# Autodesk Inventor assembly: Montagem1
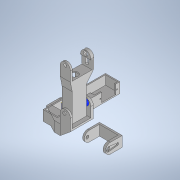
[picture p0: Inventor's stored thumbnail of the model, 180x180]
Saved by Autodesk Inventor 2022.2 (Build 262287010, 287A)
## iProperties
Created: 2022-04-04
Part Number: Montagem1
Document SubType Name: Assembly
Designer: nakai
Author: nakai
## Documents named in this file (7)
- C:\Users\nakai\Dropbox\reprap\Robo dog mini\Montagem1.iam
- C:\Users\nakai\Dropbox\reprap\Robo dog mini\ombro_base.ipt
- C:\Users\nakai\Dropbox\reprap\Robo dog mini\ombro_dir.ipt
- C:\Users\nakai\Dropbox\reprap\Robo dog mini\ombro_esq.ipt
- C:\Users\nakai\Dropbox\reprap\Robo dog mini\corpo.ipt
- C:\Users\nakai\Dropbox\reprap\Robo dog mini\servo_motor.ipt
- C:\Users\nakai\Dropbox\reprap\Robo dog mini\perna_esq.ipt
## Components (7 placed, 6 different names)
1. ombro_base:1 — Inserir:3, Inserir:4, Inserir:5
2. ombro_dir:1
3. ombro_esq:1 — Inserir:4, Inserir:5, Rotativa:1
4. corpo:1 — Inserir:1, Inserir:2, Inserir:3
5. servo_motor:1 — Inserir:1, Inserir:2
6. perna_esq:1 — Inserir:6, Inserir:7, Rotativa:1
7. servo_motor:2 — Inserir:6, Inserir:7
## Relationships (8: Insert 7, RevoluteJoint 1)
- Inserir:1: corpo:1 ↔ servo_motor:1
- Inserir:2: corpo:1 ↔ servo_motor:1
- Inserir:3: ombro_base:1 ↔ corpo:1
- Inserir:4: ombro_base:1 ↔ ombro_esq:1
- Inserir:5: ombro_base:1 ↔ ombro_esq:1
- Inserir:6: perna_esq:1 ↔ servo_motor:2
- Inserir:7: perna_esq:1 ↔ servo_motor:2
- Rotativa:1 [RevoluteJoint]: ombro_esq:1 ↔ perna_esq:1
